# Autodesk Inventor assembly: 2h
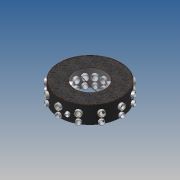
[picture p0: Inventor's stored thumbnail of the model, 180x180]
Saved by Autodesk Inventor 2014 SP1 (Build 180222100, 222)
## iProperties
Created: 2013-12-02
Part Number: 2h
Document SubType Name: Assembly
Designer: Dave
Description: Hub
Author: Dave
## Documents named in this file (9)
- C:\Users\Dave\Desktop\hera-cad\hub\hub.iam
- C:\Users\Dave\Desktop\hera-cad\hub\sonotubeInner.ipt
- C:\Users\Dave\Desktop\hera-cad\hub\sonotubeOuter.ipt
- C:\Users\Dave\Desktop\hera-cad\hub\conduit.ipt
- C:\Users\Dave\Desktop\hera-cad\hub\sleeve_sup.ipt
- C:\Users\Dave\Desktop\hera-cad\hub\rebarbar.ipt
- C:\Users\Dave\Desktop\hera-cad\hub\rebarcircle.ipt
- C:\Users\Dave\Desktop\hera-cad\hub\cement.ipt
- C:\Users\Dave\Desktop\hera-cad\hub\sleeve_spar.ipt
## Components (30 placed, 9 different names)
1. sonotubeInner:1 — Insert:1, Insert:2, Insert:5
2. sonotubeOuter:1 — Insert:1, Insert:4, Mate:2, Mate:3, Insert:6
3. rebarbar:1 — Insert:5
4. rebarcircle:1
5. cement:1 — Insert:2
6. conduit:1
7. supportSleeve — Insert:4, Mate:2
8. sleeve_sup:2
9. sleeve_sup:3
10. sleeve_sup:4
11. sleeve_sup:5
12. sleeve_sup:6
13. sleeve_sup:7
14. sleeve_sup:8
15. sleeve_sup:9
16. sleeve_sup:10
17. sleeve_sup:11
18. sleeve_sup:12
19. sleeve_spar:1 — Mate:3, Insert:6
20. sleeve_spar:2
21. sleeve_spar:3
22. sleeve_spar:4
23. sleeve_spar:5
24. sleeve_spar:6
25. sleeve_spar:7
26. sleeve_spar:8
27. sleeve_spar:9
28. sleeve_spar:10
29. sleeve_spar:11
30. sleeve_spar:12
## Component patterns: supportSleeves (12 elements), (12 elements, first: sleeve_spar:1)
## Relationships (7: Insert 5, Mate 2)
- Insert:1: sonotubeInner:1 ↔ sonotubeOuter:1
- Insert:2: sonotubeInner:1 ↔ cement:1
- Insert:4 (-271.78 mm): sonotubeOuter:1 ↔ supportSleeve
- Insert:5 (-101.6 mm): sonotubeInner:1 ↔ rebarbar:1
- Mate:2: sonotubeOuter:1 ↔ supportSleeve
- Mate:3: sonotubeOuter:1 ↔ sleeve_spar:1
- Insert:6 (-271.78 mm): sonotubeOuter:1 ↔ sleeve_spar:1
